# Autodesk Inventor assembly: EnsamblajeDodecaedro
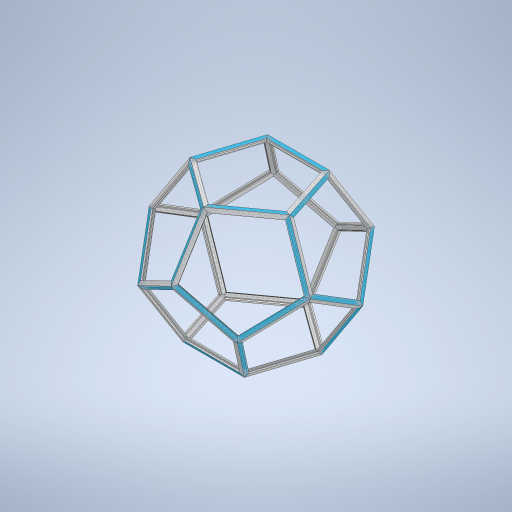
[picture p0: Inventor's stored thumbnail of the model, 512x512]
Saved by Autodesk Inventor 2024 (Build 280153000, 153)
## iProperties
Created: 2023-07-27
Part Number: EnsamblajeDodecaedro
Document SubType Name: Assembly
Designer: sergi
Author: sergi
## Documents named in this file (2)
- C:\Users\sergi\OneDrive\Escritorio\Piso\Dodecaedro\EnsamblajeDodecaedro.iam
- C:\Users\sergi\OneDrive\Escritorio\Piso\Dodecaedro\Perfil.ipt
## Components (30 placed, 1 different names)
1. Perfil:21 — Coincidencia:5, Coincidencia:6, Coincidencia:84, Coincidencia:85, Coincidencia:86
2. Perfil:22 — Coincidencia:5, Coincidencia:6, Coincidencia:13, Coincidencia:14, Coincidencia:15, Coincidencia:22
3. Perfil:24 — Coincidencia:25
4. Perfil:25 — Coincidencia:13, Coincidencia:14, Coincidencia:15, Coincidencia:23, Coincidencia:24
5. Perfil:26
6. Perfil:27 — Coincidencia:22, Coincidencia:23, Coincidencia:24
7. Perfil:28 — Coincidencia:26, Nivelación:1, Coincidencia:43, Coincidencia:44
8. Perfil:29 — Coincidencia:51, Coincidencia:52, Coincidencia:53, Coincidencia:60, Coincidencia:62
9. Perfil:30 — Coincidencia:25, Coincidencia:26, Nivelación:1, Coincidencia:33, Coincidencia:34, Coincidencia:35, Coincidencia:42
10. Perfil:31 — Coincidencia:81, Coincidencia:82, Coincidencia:83, Coincidencia:91
11. Perfil:32
12. Perfil:33 — Coincidencia:33, Coincidencia:34, Coincidencia:35
13. Perfil:34
14. Perfil:35 — Coincidencia:42, Coincidencia:43, Coincidencia:44
15. Perfil:36
16. Perfil:37
17. Perfil:38 — Coincidencia:51, Coincidencia:52, Coincidencia:53, Coincidencia:61
18. Perfil:39
19. Perfil:40 — Coincidencia:60, Coincidencia:61, Coincidencia:62
20. Perfil:41 — Coincidencia:69, Coincidencia:70, Coincidencia:71
21. Perfil:42 — Coincidencia:78, Coincidencia:79, Coincidencia:80
22. Perfil:43 — Coincidencia:87
23. Perfil:44 — Coincidencia:69, Coincidencia:70, Coincidencia:71, Coincidencia:92, Coincidencia:93, Coincidencia:94
24. Perfil:45 — Coincidencia:78, Coincidencia:79, Coincidencia:80
25. Perfil:46
26. Perfil:47
27. Perfil:48 — Coincidencia:81, Coincidencia:82, Coincidencia:83, Coincidencia:88, Coincidencia:89, Coincidencia:90
28. Perfil:49 — Coincidencia:84, Coincidencia:85, Coincidencia:86, Coincidencia:87
29. Perfil:50 — Coincidencia:88, Coincidencia:89, Coincidencia:90, Coincidencia:91
30. Perfil:51 — Coincidencia:92, Coincidencia:93, Coincidencia:94
## Relationships (87: Mate 86, Flush 1)
- Coincidencia:5 [Mate]: Perfil:21 ↔ Perfil:22
- Coincidencia:6 [Mate]: Perfil:21 ↔ Perfil:22
- [Mate]: Perfil:25 ↔ Perfil:26
- [Mate]: Perfil:25 ↔ Perfil:26
- [Mate]: Perfil:25 ↔ Perfil:26
- [Mate]: Perfil:24 ↔ Perfil:26
- [Mate]: Perfil:24 ↔ Perfil:25
- [Mate]: Perfil:24 ↔ Perfil:25
- Coincidencia:13 [Mate]: Perfil:22 ↔ Perfil:25
- Coincidencia:14 [Mate]: Perfil:22 ↔ Perfil:25
- Coincidencia:15 [Mate]: Perfil:22 ↔ Perfil:25
- [Mate]: Perfil:28 ↔ Perfil:29
- [Mate]: Perfil:28 ↔ Perfil:29
- [Mate]: Perfil:28 ↔ Perfil:29
- [Mate]: Perfil:27 ↔ Perfil:29
- [Mate]: Perfil:27 ↔ Perfil:28
- [Mate]: Perfil:27 ↔ Perfil:28
- Coincidencia:22 [Mate]: Perfil:22 ↔ Perfil:27
- Coincidencia:23 [Mate]: Perfil:25 ↔ Perfil:27
- Coincidencia:24 [Mate]: Perfil:25 ↔ Perfil:27
- Coincidencia:25 [Mate]: Perfil:24 ↔ Perfil:30
- Coincidencia:26 [Mate]: Perfil:28 ↔ Perfil:30
- Nivelación:1 [Flush]: Perfil:28 ↔ Perfil:30
- [Mate]: Perfil:32 ↔ Perfil:33
- [Mate]: Perfil:32 ↔ Perfil:33
- [Mate]: Perfil:32 ↔ Perfil:33
- [Mate]: Perfil:31 ↔ Perfil:33
- [Mate]: Perfil:31 ↔ Perfil:32
- [Mate]: Perfil:31 ↔ Perfil:32
- Coincidencia:33 [Mate]: Perfil:30 ↔ Perfil:33
- Coincidencia:34 [Mate]: Perfil:30 ↔ Perfil:33
- Coincidencia:35 [Mate]: Perfil:30 ↔ Perfil:33
- [Mate]: Perfil:35 ↔ Perfil:36
- [Mate]: Perfil:35 ↔ Perfil:36
- [Mate]: Perfil:35 ↔ Perfil:36
- [Mate]: Perfil:34 ↔ Perfil:36
- [Mate]: Perfil:34 ↔ Perfil:35
- [Mate]: Perfil:34 ↔ Perfil:35
- Coincidencia:42 [Mate]: Perfil:30 ↔ Perfil:35
- Coincidencia:43 [Mate]: Perfil:28 ↔ Perfil:35
- Coincidencia:44 [Mate]: Perfil:28 ↔ Perfil:35
- [Mate]: Perfil:37 ↔ Perfil:38
- [Mate]: Perfil:37 ↔ Perfil:38
- Coincidencia:51 [Mate]: Perfil:29 ↔ Perfil:38
- Coincidencia:52 [Mate]: Perfil:29 ↔ Perfil:38
- Coincidencia:53 [Mate]: Perfil:29 ↔ Perfil:38
- [Mate]: Perfil:40 ↔ Perfil:41
- [Mate]: Perfil:40 ↔ Perfil:41
- [Mate]: Perfil:40 ↔ Perfil:41
- [Mate]: Perfil:39 ↔ Perfil:41
- [Mate]: Perfil:39 ↔ Perfil:40
- [Mate]: Perfil:39 ↔ Perfil:40
- Coincidencia:60 [Mate]: Perfil:29 ↔ Perfil:40
- Coincidencia:61 [Mate]: Perfil:38 ↔ Perfil:40
- Coincidencia:62 [Mate]: Perfil:29 ↔ Perfil:40
- [Mate]: Perfil:43 ↔ Perfil:44
- [Mate]: Perfil:43 ↔ Perfil:44
- [Mate]: Perfil:43 ↔ Perfil:44
- [Mate]: Perfil:42 ↔ Perfil:44
- [Mate]: Perfil:42 ↔ Perfil:43
- [Mate]: Perfil:42 ↔ Perfil:43
- Coincidencia:69 [Mate]: Perfil:41 ↔ Perfil:44
- Coincidencia:70 [Mate]: Perfil:41 ↔ Perfil:44
- Coincidencia:71 [Mate]: Perfil:41 ↔ Perfil:44
- [Mate]: Perfil:46 ↔ Perfil:47
- [Mate]: Perfil:46 ↔ Perfil:47
- [Mate]: Perfil:46 ↔ Perfil:47
- [Mate]: Perfil:45 ↔ Perfil:47
- [Mate]: Perfil:45 ↔ Perfil:46
- [Mate]: Perfil:45 ↔ Perfil:46
- Coincidencia:78 [Mate]: Perfil:42 ↔ Perfil:45
- Coincidencia:79 [Mate]: Perfil:42 ↔ Perfil:45
- Coincidencia:80 [Mate]: Perfil:42 ↔ Perfil:45
- Coincidencia:81 [Mate]: Perfil:31 ↔ Perfil:48
- Coincidencia:82 [Mate]: Perfil:31 ↔ Perfil:48
- Coincidencia:83 [Mate]: Perfil:31 ↔ Perfil:48
- Coincidencia:84 [Mate]: Perfil:21 ↔ Perfil:49
- Coincidencia:85 [Mate]: Perfil:21 ↔ Perfil:49
- Coincidencia:86 [Mate]: Perfil:21 ↔ Perfil:49
- Coincidencia:87 [Mate]: Perfil:43 ↔ Perfil:49
- Coincidencia:88 [Mate]: Perfil:48 ↔ Perfil:50
- Coincidencia:89 [Mate]: Perfil:48 ↔ Perfil:50
- Coincidencia:90 [Mate]: Perfil:48 ↔ Perfil:50
- Coincidencia:91 [Mate]: Perfil:31 ↔ Perfil:50
- Coincidencia:92 [Mate]: Perfil:44 ↔ Perfil:51
- Coincidencia:93 [Mate]: Perfil:44 ↔ Perfil:51
- Coincidencia:94 [Mate]: Perfil:44 ↔ Perfil:51
## Named parameters: d6_d0 = 0 mm, d7_d1 = 0 mm, d8_d2 = 0 mm, d9_d3 = 0 mm, d10_d4 = 0 mm, d11_d5 = 0 mm, d17_d0 = 0 mm, d18_d1 = 0 mm, d19_d2 = 0 mm, d20_d3 = 0 mm, d21_d4 = 0 mm, d22_d5 = 0 mm, d29_d0 = 0 mm, d30_d1 = 0 mm, d31_d2 = 0 mm, d32_d3 = 0 mm, d33_d4 = 0 mm, d34_d5 = 0 mm, d38_d0 = 0 mm, d39_d1 = 0 mm, d40_d2 = 0 mm, d41_d3 = 0 mm, d42_d4 = 0 mm, d43_d5 = 0 mm, d51_d4 = 0 mm, d52_d5 = 0 mm, d56_d0 = 0 mm, d57_d1 = 0 mm, d58_d2 = 0 mm, d59_d3 = 0 mm, d60_d4 = 0 mm, d61_d5 = 0 mm, d65_d29_d0 = 0 mm, d66_d30_d1 = 0 mm, d67_d31_d2 = 0 mm, d68_d32_d3 = 0 mm, d69_d33_d4 = 0 mm, d70_d34_d5 = 0 mm, d74_d29_d0 = 0 mm, d75_d30_d1 = 0 mm, d76_d31_d2 = 0 mm, d77_d32_d3 = 0 mm, d78_d33_d4 = 0 mm, d79_d34_d5 = 0 mm
